# Autodesk Inventor assembly: case
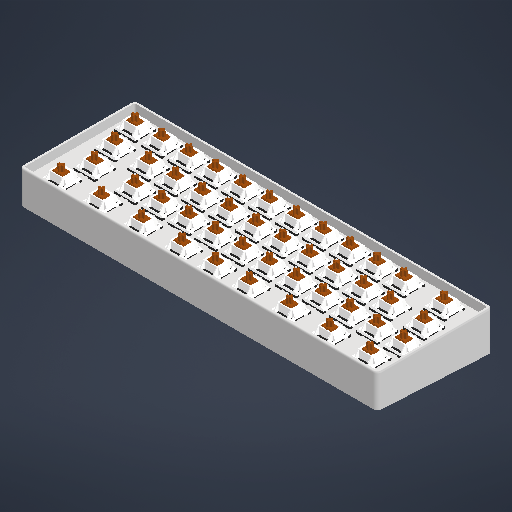
[picture p0: Inventor's stored thumbnail of the model, 512x512]
Saved by Autodesk Inventor 2026 (Build 300175050, 175E)
## iProperties
Created: 2025-06-14
Part Number: case
Document SubType Name: Assembly
Designer: nikla
Author: nikla
## Documents named in this file (4)
- C:\Users\nikla\git\40percent\case\case.iam
- C:\Users\nikla\git\40percent\40percent\40percent\40percent\40percent.iam
- C:\Users\nikla\git\40percent\case\Top.ipt
- C:\Users\nikla\git\40percent\case\Bottom.ipt
## Components (3 placed, 3 different names)
1. 40percent:1 [sub-assembly] — Fluchtend:1, Fluchtend:2
2. Top:1 — Fluchtend:1
3. Bottom:1 — Fluchtend:2
## Relationships (2: Flush 2)
- Fluchtend:1 [Flush]: 40percent:1 ↔ Top:1
- Fluchtend:2 [Flush]: 40percent:1 ↔ Bottom:1
